# Autodesk Inventor assembly: Final_Boss
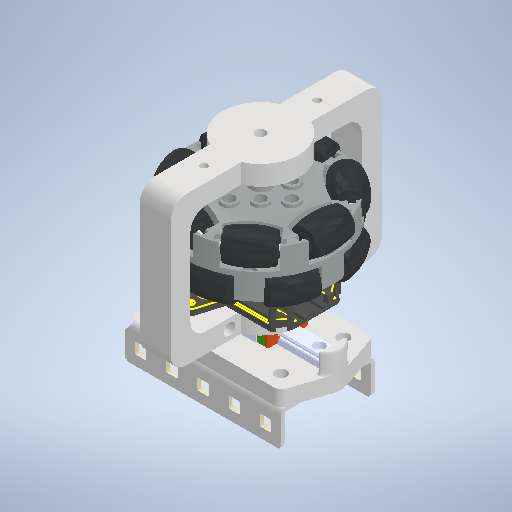
[picture p0: Inventor's stored thumbnail of the model, 512x512]
Saved by Autodesk Inventor 2025.1 (Build 291241020, 241B)
## iProperties
Created: 2024-11-26
Part Number: Final_Boss
Document SubType Name: Assembly
Designer: AtuStem
Author: AtuStem
## Documents named in this file (9)
- C:\Users\AtuStem\Documents\GitHub\ATUM-V5RC-High-Stakes-CAD\Odometers_Collin\Final_Boss.iam
- C:\Users\AtuStem\Documents\GitHub\ATUM-V5RC-High-Stakes-CAD\Odometers_Collin\Linear Rail Files\LinearRail-LWL7B-100mm\LinearRail-LWL7B-100mm\LinearRail-LWL7B-100mm.ipt
- C:\Users\AtuStem\Documents\GitHub\ATUM-V5RC-High-Stakes-CAD\Odometers_Collin\Linear_Odom.ipt
- C:\Users\AtuStem\Documents\GitHub\ATUM-V5RC-High-Stakes-CAD\Odometers_Collin\Linear Rail Files\Carriage-LWL7B\Carriage-LWL7B\Carriage-LWL7B.ipt
- C:\Users\AtuStem\Documents\GitHub\ATUM-V5RC-High-Stakes-CAD\Odometers_Collin\Encoder_Base.ipt
- C:\Users\AtuStem\Documents\GitHub\ATUM-V5RC-High-Stakes-CAD\VEX-CAD-Inventor\Motion\Insert Circle.ipt
- C:\Users\AtuStem\Documents\GitHub\ATUM-V5RC-High-Stakes-CAD\Odometers_Collin\IQ_OMNI.iam
- C:\Users\AtuStem\Documents\GitHub\ATUM-V5RC-High-Stakes-CAD\Odometers_Collin\Linear_Mount.ipt
- C:\Users\AtuStem\Documents\GitHub\ATUM-V5RC-High-Stakes-CAD\VEX-CAD-Inventor\Structure\C Channel\Aluminum 1x3x1\Alu C 1x3x1x5.ipt
## Components (9 placed, 8 different names)
1. LinearRail-LWL7B-100mm:1 — Mate:9, Mate:10, Mate:12, Mate:13
2. Linear_Odom:1 — Mate:1, Mate:2, Mate:3, Mate:4, Mate:5, Mate:6, Flush:1, Flush:2, Mate:11, Flush:3
3. Carriage-LWL7B:1 — Mate:1, Mate:2, Mate:3, Mate:9, Mate:10
4. Encoder_Base:1 — Mate:4, Mate:5, Mate:6, Mate:7
5. Insert Circle:1 — Flush:1, Mate:7, Mate:8
6. Insert Circle:2 — Flush:2, Mate:8, Flush:3
7. IQ_OMNI:1 [sub-assembly] — Mate:11
8. Linear_Mount:1 — Mate:12, Mate:13, Mate:14, Mate:15
9. Alu C 1x3x1x5:1 — Mate:14, Mate:15
## Relationships (18: Mate 15, Flush 3)
- Mate:1: Linear_Odom:1 ↔ Carriage-LWL7B:1
- Mate:2: Linear_Odom:1 ↔ Carriage-LWL7B:1
- Mate:3: Linear_Odom:1 ↔ Carriage-LWL7B:1
- Mate:4: Linear_Odom:1 ↔ Encoder_Base:1
- Mate:5: Linear_Odom:1 ↔ Encoder_Base:1
- Mate:6: Linear_Odom:1 ↔ Encoder_Base:1
- Flush:1: Linear_Odom:1 ↔ Insert Circle:1
- Mate:7: Encoder_Base:1 ↔ Insert Circle:1
- Flush:2: Linear_Odom:1 ↔ Insert Circle:2
- Mate:8: Insert Circle:1 ↔ Insert Circle:2
- Mate:9: LinearRail-LWL7B-100mm:1 ↔ Carriage-LWL7B:1
- Mate:10 (0.2032 mm): LinearRail-LWL7B-100mm:1 ↔ Carriage-LWL7B:1
- Mate:11: Linear_Odom:1 ↔ IQ_OMNI:1
- Flush:3: Linear_Odom:1 ↔ Insert Circle:2
- Mate:12: LinearRail-LWL7B-100mm:1 ↔ Linear_Mount:1
- Mate:13: LinearRail-LWL7B-100mm:1 ↔ Linear_Mount:1
- Mate:14: Linear_Mount:1 ↔ Alu C 1x3x1x5:1
- Mate:15: Linear_Mount:1 ↔ Alu C 1x3x1x5:1
